# Autodesk Inventor assembly: Assembly1
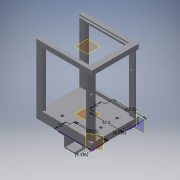
[picture p0: Inventor's stored thumbnail of the model, 180x180]
Saved by Autodesk Inventor 2016 (Build 200138000, 138)
## iProperties
Created: 2018-10-15
Part Number: Assembly1
Document SubType Name: Assembly
Designer: Kyle
Author: Kyle
## Documents named in this file (3)
- A:\Inventor current projects\PacBot\V0.5.0\Assembly1.iam
- A:\Inventor current projects\PacBot\V0.5.0\Base.ipt
- A:\Inventor current projects\PacBot\V0.5.0\Motor_shroud.ipt
## Components (3 placed, 2 different names)
1. Base:1 — Mate:1, Flush:1, Flush:2, Mate:2, Flush:3, Flush:4
2. Motor_shroud:1 — Mate:1, Flush:1, Flush:2
3. Motor_shroud:2 — Mate:2, Flush:3, Flush:4
## Relationships (6: Flush 4, Mate 2)
- Mate:1: Base:1 ↔ Motor_shroud:1
- Flush:1: Base:1 ↔ Motor_shroud:1
- Flush:2: Base:1 ↔ Motor_shroud:1
- Mate:2: Base:1 ↔ Motor_shroud:2
- Flush:3: Base:1 ↔ Motor_shroud:2
- Flush:4: Base:1 ↔ Motor_shroud:2
